# Autodesk Inventor assembly: x_motor_assembly
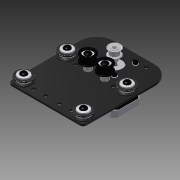
[picture p0: Inventor's stored thumbnail of the model, 180x180]
Saved by Autodesk Inventor 2014 (Build 180170000, 170)
## iProperties
Created: 2013-07-18
Part Number: x_motor_assembly
Document SubType Name: Assembly
Designer: Edward
Author: Edward
## Documents named in this file (14)
- C:\Users\Edward\Documents\GitHub\Shapeoko_Experimental\Shapeoko_CP\Autodesk_Inventor_Project\x_motor_assembly.iam
- C:\Users\Edward\Documents\GitHub\Shapeoko_Experimental\Shapeoko_CP\Autodesk_Inventor_Project\x_motor_mount_v2.ipt
- C:\Users\Edward\Documents\GitHub\Shapeoko_Experimental\Shapeoko_CP\Autodesk_Inventor_Project\B30037.iam
- C:\Users\Edward\Documents\GitHub\Shapeoko_Experimental\Shapeoko_CP\Autodesk_Inventor_Project\SM-H03.ipt
- C:\Users\Edward\Documents\GitHub\Shapeoko_Experimental\Shapeoko_CP\Autodesk_Inventor_Project\91239A233.ipt
- C:\Users\Edward\Documents\GitHub\Shapeoko_Experimental\Shapeoko_CP\Autodesk_Inventor_Project\SM-H04.ipt
- C:\Users\Edward\Documents\GitHub\Shapeoko_Experimental\Shapeoko_CP\Autodesk_Inventor_Project\B18033.ipt
- C:\Users\Edward\Documents\GitHub\Shapeoko_Experimental\Shapeoko_CP\Autodesk_Inventor_Project\M1173041- NEMA 17.ipt
- C:\Users\Edward\Documents\GitHub\Shapeoko_Experimental\Shapeoko_CP\Autodesk_Inventor_Project\a_6a51-020df0606.ipt
- C:\Users\Edward\Documents\GitHub\Shapeoko_Experimental\Shapeoko_CP\Autodesk_Inventor_Project\91290A113.ipt
- C:\Users\Edward\Documents\GitHub\Shapeoko_Experimental\Shapeoko_CP\Autodesk_Inventor_Project\91166A210.ipt
- C:\Users\Edward\Documents\GitHub\Shapeoko_Experimental\Shapeoko_CP\Autodesk_Inventor_Project\B30041.iam
- C:\Users\Edward\Documents\GitHub\Shapeoko_Experimental\Shapeoko_CP\Autodesk_Inventor_Project\91239A236.ipt
- C:\Users\Edward\Documents\GitHub\Shapeoko_Experimental\Shapeoko_CP\Autodesk_Inventor_Project\AS38-12-20.ipt
## Components (41 placed, 13 different names)
1. x_motor_mount_v2:1 — Insert:7, Insert:8, Insert:9, Insert:10, Insert:13, Insert:16, Mate:3, Mate:4, Insert:19, Mate:6, Insert:20, Insert:24, Insert:25, Insert:26, Insert:31, Insert:32, Insert:37, Insert:38
2. B30037:1 [sub-assembly]
3. SM-H03:1 — Insert:7
4. 91239A233:1
5. SM-H04:1
6. SM-H03:2 — Insert:9
7. B30037:2 [sub-assembly]
8. SM-H03:3 — Insert:8
9. 91239A233:2
10. SM-H04:2
11. SM-H03:4 — Insert:10
12. B18033:1 — Insert:13
13. SM-H03:5 — Mate:4
14. 91239A233:3
15. B30037:3 [sub-assembly]
16. B18033:2 — Insert:16
17. SM-H03:6 — Mate:3
18. 91239A233:4
19. B30037:4 [sub-assembly]
20. M1173041- NEMA 17:1 — Insert:19, Mate:6
21. a_6a51-020df0606:1
22. 91290A113:1
23. 91166A210:1 — Insert:20
24. 91290A113:2
25. 91166A210:2 — Insert:26
26. 91290A113:3
27. 91166A210:3 — Insert:25
28. 91290A113:4
29. 91166A210:4 — Insert:24
30. B30041:1 [sub-assembly]
31. 91239A236:1
32. AS38-12-20:1
33. SM-H03:7 — Insert:31
34. SM-H04:3
35. SM-H03:8 — Insert:32
36. B30041:2 [sub-assembly]
37. 91239A236:2
38. AS38-12-20:2
39. SM-H03:9 — Insert:37
40. SM-H04:4
41. SM-H03:10 — Insert:38
## Relationships (44: Insert 38, Mate 6)
- [Insert]: B30037:1 ↔ SM-H03:1
- [Insert]: B30037:1 ↔ 91239A233:1
- [Insert]: SM-H04:1 ↔ SM-H03:2
- [Insert]: B30037:2 ↔ SM-H03:3
- [Insert]: B30037:2 ↔ 91239A233:2
- [Insert]: SM-H04:2 ↔ SM-H03:4
- Insert:7: x_motor_mount_v2:1 ↔ SM-H03:1
- Insert:8: x_motor_mount_v2:1 ↔ SM-H03:3
- Insert:9: x_motor_mount_v2:1 ↔ SM-H03:2
- Insert:10: x_motor_mount_v2:1 ↔ SM-H03:4
- [Insert]: SM-H03:5 ↔ B30037:3
- [Insert]: 91239A233:3 ↔ B30037:3
- [Mate]: B18033:1 ↔ 91239A233:3
- Insert:13: x_motor_mount_v2:1 ↔ B18033:1
- [Insert]: SM-H03:6 ↔ B30037:4
- [Insert]: 91239A233:4 ↔ B30037:4
- [Mate]: B18033:2 ↔ 91239A233:4
- Insert:16: x_motor_mount_v2:1 ↔ B18033:2
- Mate:3: x_motor_mount_v2:1 ↔ SM-H03:6
- Mate:4: x_motor_mount_v2:1 ↔ SM-H03:5
- [Mate]: M1173041- NEMA 17:1 ↔ a_6a51-020df0606:1
- [Insert]: M1173041- NEMA 17:1 ↔ a_6a51-020df0606:1
- [Insert]: 91290A113:1 ↔ 91166A210:1
- Insert:19: x_motor_mount_v2:1 ↔ M1173041- NEMA 17:1
- Mate:6: x_motor_mount_v2:1 ↔ M1173041- NEMA 17:1
- Insert:20: x_motor_mount_v2:1 ↔ 91166A210:1
- [Insert]: 91290A113:2 ↔ 91166A210:2
- [Insert]: 91290A113:3 ↔ 91166A210:3
- [Insert]: 91290A113:4 ↔ 91166A210:4
- Insert:24: x_motor_mount_v2:1 ↔ 91166A210:4
- Insert:25: x_motor_mount_v2:1 ↔ 91166A210:3
- Insert:26: x_motor_mount_v2:1 ↔ 91166A210:2
- [Insert]: B30041:1 ↔ 91239A236:1
- [Insert]: B30041:1 ↔ AS38-12-20:1
- [Insert]: AS38-12-20:1 ↔ SM-H03:7
- [Insert]: SM-H04:3 ↔ SM-H03:8
- Insert:31: x_motor_mount_v2:1 ↔ SM-H03:7
- Insert:32: x_motor_mount_v2:1 ↔ SM-H03:8
- [Insert]: B30041:2 ↔ 91239A236:2
- [Insert]: B30041:2 ↔ AS38-12-20:2
- [Insert]: AS38-12-20:2 ↔ SM-H03:9
- [Insert]: SM-H04:4 ↔ SM-H03:10
- Insert:37: x_motor_mount_v2:1 ↔ SM-H03:9
- Insert:38: x_motor_mount_v2:1 ↔ SM-H03:10
## Named parameters: d17_d1 = 0 mm, d18_d7 = 0 mm, d3_d17_d1 = 0 mm, d4_d18_d7 = 0 mm, d5_d9 = 0 mm, d11_d10 = 0 mm, d22_d12 = 0 mm, d15_d10 = 0 mm, d16_d11 = 0 mm, d17_d22_d12 = 0 mm, d182_d39 = 0 mm, d27_d182_d39 = 0 mm, d28_d182_d39 = 0 mm, d29_d182_d39 = 0 mm, d33_d32 = 0 mm, d36_d9 = 0 mm, d40_d32 = 0 mm, d41_d35 = 0 mm, d42_d49 = 0 mm, d43_d36_d9 = 0 mm
